# Autodesk Inventor assembly: ASY APN FDS way3
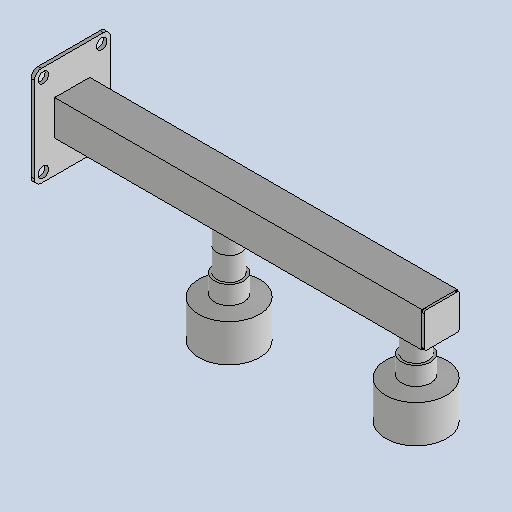
[picture p0: Inventor's stored thumbnail of the model, 512x512]
Saved by Autodesk Inventor 2025.1 (Build 291241020, 241B)
## iProperties
Created: 2025-07-02
Part Number: ASY APN FDS way3
Document SubType Name: Assembly
Designer: user
Author: user
## Documents named in this file (7)
- C:\Users\admin\Yandex.Disk\home pc\Inventor\ANP-Antipayuta\ASY APN FDS way3.iam
- C:\Users\admin\Yandex.Disk\home pc\Inventor\ANP-Antipayuta\APN 756 FDS 1200 way tube 3.ipt
- C:\Users\admin\Yandex.Disk\home pc\Inventor\ANP-Antipayuta\APN dummy filter element.ipt
- C:\Users\admin\Yandex.Disk\home pc\Inventor\ANP-Antipayuta\APN dummy pipe nippel.ipt
- C:\Users\admin\Yandex.Disk\home pc\Inventor\ANP-Antipayuta\APN 1757 FDS 1200 way tube 7.ipt
- C:\Users\admin\Yandex.Disk\home pc\Inventor\ANP-Antipayuta\APN 760 FDS 1200 FLANGE 3.ipt
- C:\Users\admin\Yandex.Disk\home pc\Inventor\ANP-Antipayuta\APN 766 FDS 1200 CUP 1.ipt
## Components (8 placed, 6 different names)
1. PNS 756 FDS 1200 way tube 3.ipt:1 — Rigid:7
2. PNS dummy filter element.ipt:1
3. PNS dummy pipe nippel.ipt:1
4. PNS 759 FDS 1200 way tube 7.ipt:1
5. PNS dummy filter element.ipt:2
6. PNS dummy pipe nippel.ipt:2
7. PNS 760 FDS 1200 FLANGE 3.ipt:1
8. PNS 766 FDS 1200 CUP 1.ipt:1 — Rigid:7
## Relationships (7: WeldJoint 7)
- [WeldJoint]: PNS dummy filter element.ipt:1 ↔ PNS dummy pipe nippel.ipt:1
- [WeldJoint]: PNS 756 FDS 1200 way tube 3.ipt:1 ↔ PNS dummy pipe nippel.ipt:1
- [WeldJoint]: PNS dummy filter element.ipt:2 ↔ PNS dummy pipe nippel.ipt:2
- [WeldJoint]: PNS 759 FDS 1200 way tube 7.ipt:1 ↔ PNS dummy pipe nippel.ipt:2
- [WeldJoint]: PNS 756 FDS 1200 way tube 3.ipt:1 ↔ PNS 759 FDS 1200 way tube 7.ipt:1
- [WeldJoint] (-3 mm): PNS 756 FDS 1200 way tube 3.ipt:1 ↔ PNS 760 FDS 1200 FLANGE 3.ipt:1
- Rigid:7 [WeldJoint]: PNS 756 FDS 1200 way tube 3.ipt:1 ↔ PNS 766 FDS 1200 CUP 1.ipt:1
## Named parameters: d34_d31 = 0 mm, d45_d43_d40_d37_d34_d31 = 0 mm
